# Autodesk Inventor assembly: Solarbotics_GM9-Assem
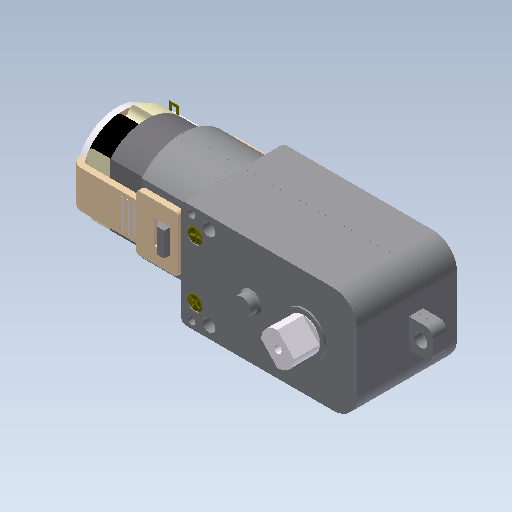
[picture p0: Inventor's stored thumbnail of the model, 512x512]
Saved by Autodesk Inventor 2020.1 (Build 241239000, 239)
## iProperties
Created: 2013-04-22
Part Number: Solarbotics_GM9-Assem
Document SubType Name: Assembly
Designer: justin
## Documents named in this file (7)
- C:\Users\amirs\Downloads\Solarbotics_GM9-Assem.iam
- C:\Users\amirs\Downloads\GM9-driver_side.ipt
- C:\Users\amirs\Downloads\GM9-encoder_side.ipt
- C:\Users\amirs\Downloads\RM3-regular motor.ipt
- C:\Users\amirs\Downloads\GMstrap2.ipt
- C:\Users\amirs\Downloads\screw_head1.ipt
- C:\Users\amirs\Downloads\output shaft.ipt
## Components (7 placed, 6 different names)
1. GM9-driver_side:1 — Flush:3, Insert:1, Mate:1, Mate:2, Flush:7, Flush:8
2. GM9-encoder_side:1 — Flush:1, Flush:2
3. RM3-regular motor:1 — Flush:4, Angle:1, Angle:2, Flush:5, Flush:6
4. GMstrap2:1 — Flush:1, Flush:2, Flush:3, Flush:4, Angle:1, Angle:2, Flush:5, Flush:6
5. screw_head1:1 — Mate:2, Flush:7
6. screw_head1:2 — Mate:1, Flush:8
7. output shaft:1 — Insert:1
## Relationships (13: Flush 8, Angle 2, Mate 2, Insert 1)
- Flush:1 (-1.6256 mm): GM9-encoder_side:1 ↔ GMstrap2:1
- Flush:2 (40.1066 mm): GM9-encoder_side:1 ↔ GMstrap2:1
- Flush:3 (7.239 mm): GM9-driver_side:1 ↔ GMstrap2:1
- Flush:4 (0.7366 mm): RM3-regular motor:1 ↔ GMstrap2:1
- Angle:1 (0 deg): RM3-regular motor:1 ↔ GMstrap2:1
- Angle:2 (0 deg): RM3-regular motor:1 ↔ GMstrap2:1
- Flush:5 (-0.127 mm): RM3-regular motor:1 ↔ GMstrap2:1
- Flush:6 (2.7178 mm): RM3-regular motor:1 ↔ GMstrap2:1
- Insert:1: GM9-driver_side:1 ↔ output shaft:1
- Mate:1: GM9-driver_side:1 ↔ screw_head1:2
- Mate:2: GM9-driver_side:1 ↔ screw_head1:1
- Flush:7: GM9-driver_side:1 ↔ screw_head1:1
- Flush:8: GM9-driver_side:1 ↔ screw_head1:2
